# Autodesk Inventor assembly: Table Assembly
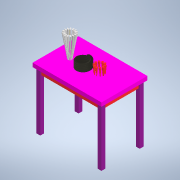
[picture p0: Inventor's stored thumbnail of the model, 180x180]
Saved by Autodesk Inventor 2022.4 (Build 264492000, 492)
## iProperties
Created: 2024-05-02
Part Number: Table Assembly
Document SubType Name: Assembly
Designer: t60147996
Author: t60147996
## Documents named in this file (8)
- D:\Spring 2024\Advanced CAD\Table\Table Assembly.iam
- D:\Spring 2024\Advanced CAD\Table\Table Leg.ipt
- D:\Spring 2024\Advanced CAD\Table\Table Short Rail.ipt
- D:\Spring 2024\Advanced CAD\Table\Table Long Rail.ipt
- D:\Spring 2024\Advanced CAD\Table\Table Top.ipt
- D:\Spring 2024\Advanced CAD\Table\Table Decoration 1.ipt
- D:\Spring 2024\Advanced CAD\Table\Table Decoration 2.ipt
- D:\Spring 2024\Advanced CAD\Table\Table Decoration 3.ipt
## Components (12 placed, 7 different names)
1. Table Leg:1 — Mate:5, Flush:2, Flush:3, Mate:9, Mate:13, Flush:12
2. Table Leg:2 — Mate:7, Mate:8, Flush:4, Flush:5, Mate:10, Flush:8, Mate:14, Flush:11
3. Table Leg:3 — Mate:1, Mate:4, Flush:1, Flush:9, Mate:12
4. Table Leg:4 — Mate:2, Mate:6, Flush:6, Flush:7, Mate:11, Flush:10
5. Table Short Rail:1 — Mate:4, Mate:5, Flush:1, Flush:2, Mate:12
6. Table Short Rail:2 — Mate:6, Mate:7, Flush:5, Mate:10, Flush:10, Mate:14
7. Table Long Rail:1 — Mate:1, Mate:2, Flush:7, Mate:11, Flush:9
8. Table Long Rail:2 — Mate:8, Flush:3, Flush:4, Flush:6, Flush:8, Mate:13
9. Table Top:1 — Mate:9, Flush:11, Flush:12, Mate:15, Mate:16, Mate:17
10. Table Decoration 1:1 — Mate:15
11. Table Decoration 2:1 — Mate:17
12. Table Decoration 3:1 — Mate:16
## Relationships (28: Mate 16, Flush 12)
- Mate:1: Table Leg:3 ↔ Table Long Rail:1
- Mate:2: Table Leg:4 ↔ Table Long Rail:1
- Mate:4: Table Leg:3 ↔ Table Short Rail:1
- Mate:5: Table Leg:1 ↔ Table Short Rail:1
- Mate:6: Table Leg:4 ↔ Table Short Rail:2
- Mate:7: Table Leg:2 ↔ Table Short Rail:2
- Mate:8: Table Leg:2 ↔ Table Long Rail:2
- Flush:1: Table Leg:3 ↔ Table Short Rail:1
- Flush:2: Table Leg:1 ↔ Table Short Rail:1
- Flush:3: Table Leg:1 ↔ Table Long Rail:2
- Flush:4: Table Leg:2 ↔ Table Long Rail:2
- Flush:5: Table Leg:2 ↔ Table Short Rail:2
- Flush:6: Table Leg:4 ↔ Table Long Rail:2
- Flush:7: Table Leg:4 ↔ Table Long Rail:1
- Mate:9: Table Leg:1 ↔ Table Top:1
- Mate:10: Table Leg:2 ↔ Table Short Rail:2
- Flush:8: Table Leg:2 ↔ Table Long Rail:2
- Mate:11: Table Leg:4 ↔ Table Long Rail:1
- Flush:9: Table Leg:3 ↔ Table Long Rail:1
- Mate:12: Table Leg:3 ↔ Table Short Rail:1
- Mate:13: Table Leg:1 ↔ Table Long Rail:2
- Flush:10: Table Leg:4 ↔ Table Short Rail:2
- Mate:14: Table Leg:2 ↔ Table Short Rail:2
- Flush:11 (-25.4 mm): Table Leg:2 ↔ Table Top:1
- Flush:12 (-25.4 mm): Table Leg:1 ↔ Table Top:1
- Mate:15: Table Top:1 ↔ Table Decoration 1:1
- Mate:16: Table Top:1 ↔ Table Decoration 3:1
- Mate:17: Table Top:1 ↔ Table Decoration 2:1
